# Autodesk Inventor assembly: RobotAsem
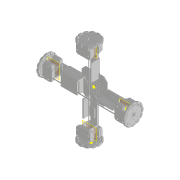
[picture p0: Inventor's stored thumbnail of the model, 180x180]
Saved by Autodesk Inventor 2022 (Build 260153000, 153)
## iProperties
Created: 2022-10-20
Part Number: RobotAsem
Document SubType Name: Assembly
Designer: MVeszpremi
Author: MVeszpremi
## Documents named in this file (8)
- C:\Users\veszp\Dropbox\180DAB CAD\RobotAsem.iam
- C:\Users\veszp\Dropbox\180DAB CAD\RobotBase.ipt
- C:\Users\veszp\Dropbox\180DAB CAD\StepperMotorHolder.ipt
- C:\Users\veszp\Dropbox\180DAB CAD\RobotBaseMotorExt.ipt
- C:\Users\veszp\Dropbox\180DAB CAD\Placeholde_stepperdriverr.ipt
- C:\Users\veszp\Dropbox\180DAB CAD\Wheel.ipt
- C:\Users\veszp\Dropbox\180DAB CAD\BaseStabilizerAttachment.ipt
- C:\Users\veszp\Dropbox\180DAB CAD\Paceholder_shaft.ipt
## Components (20 placed, 7 different names)
1. RobotBase:1 — Mate:1, Mate:2, Mate:3, Mate:4, Mate:5, Mate:6, Mate:7, Mate:8, Mate:9, Mate:10, Mate:11, Mate:12
2. RobotBaseMotorExt:1 — Mate:1, Mate:2, Mate:3, Mate:25, Mate:26, Mate:36, Mate:37, Mate:38
3. RobotBaseMotorExt:2 — Mate:4, Mate:5, Mate:6, Mate:27, Mate:28, Mate:29
4. RobotBaseMotorExt:3 — Mate:7, Mate:8, Mate:9, Mate:33, Mate:34, Mate:35
5. RobotBaseMotorExt:4 — Mate:10, Mate:11, Mate:12, Mate:30, Mate:31, Mate:32
6. Placeholde_stepperdriverr:1 — Mate:25, Mate:26
7. StepperMotorHolder:1 — Mate:27, Mate:28, Mate:29, Mate:43, Mate:44, Mate:45, Mate:46
8. StepperMotorHolder:2 — Mate:30, Mate:31, Mate:32, Mate:41, Mate:47, Mate:48, Mate:49
9. StepperMotorHolder:3 — Mate:33, Mate:34, Mate:35, Mate:42, Mate:50, Mate:51, Mate:52
10. StepperMotorHolder:4 — Mate:36, Mate:37, Mate:38, Mate:39, Mate:40, Mate:53, Mate:54, Mate:55
11. Wheel:1 — Mate:39, Mate:40
12. Wheel:2 — Mate:41
13. Wheel:3 — Mate:42
14. Wheel:4 — Mate:43
15. BaseStabilizerAttachment:1 — Mate:44, Mate:45, Mate:46, Mate:58
16. BaseStabilizerAttachment:2 — Mate:47, Mate:48, Mate:49, Mate:59
17. BaseStabilizerAttachment:3 — Mate:50, Mate:51, Mate:52, Mate:57
18. BaseStabilizerAttachment:4 — Mate:53, Mate:54, Mate:55, Mate:56
19. Paceholder_shaft:1 — Mate:56, Mate:57
20. Paceholder_shaft:2 — Mate:58, Mate:59
## Relationships (47: Mate 47)
- Mate:1: RobotBase:1 ↔ RobotBaseMotorExt:1
- Mate:2: RobotBase:1 ↔ RobotBaseMotorExt:1
- Mate:3: RobotBase:1 ↔ RobotBaseMotorExt:1
- Mate:4: RobotBase:1 ↔ RobotBaseMotorExt:2
- Mate:5: RobotBase:1 ↔ RobotBaseMotorExt:2
- Mate:6: RobotBase:1 ↔ RobotBaseMotorExt:2
- Mate:7: RobotBase:1 ↔ RobotBaseMotorExt:3
- Mate:8: RobotBase:1 ↔ RobotBaseMotorExt:3
- Mate:9: RobotBase:1 ↔ RobotBaseMotorExt:3
- Mate:10: RobotBase:1 ↔ RobotBaseMotorExt:4
- Mate:11: RobotBase:1 ↔ RobotBaseMotorExt:4
- Mate:12: RobotBase:1 ↔ RobotBaseMotorExt:4
- Mate:25: RobotBaseMotorExt:1 ↔ Placeholde_stepperdriverr:1
- Mate:26 (6.5 mm): RobotBaseMotorExt:1 ↔ Placeholde_stepperdriverr:1
- Mate:27: RobotBaseMotorExt:2 ↔ StepperMotorHolder:1
- Mate:28: RobotBaseMotorExt:2 ↔ StepperMotorHolder:1
- Mate:29: RobotBaseMotorExt:2 ↔ StepperMotorHolder:1
- Mate:30: RobotBaseMotorExt:4 ↔ StepperMotorHolder:2
- Mate:31: RobotBaseMotorExt:4 ↔ StepperMotorHolder:2
- Mate:32: RobotBaseMotorExt:4 ↔ StepperMotorHolder:2
- Mate:33: RobotBaseMotorExt:3 ↔ StepperMotorHolder:3
- Mate:34: RobotBaseMotorExt:3 ↔ StepperMotorHolder:3
- Mate:35: RobotBaseMotorExt:3 ↔ StepperMotorHolder:3
- Mate:36: RobotBaseMotorExt:1 ↔ StepperMotorHolder:4
- Mate:37: RobotBaseMotorExt:1 ↔ StepperMotorHolder:4
- Mate:38: RobotBaseMotorExt:1 ↔ StepperMotorHolder:4
- Mate:39: StepperMotorHolder:4 ↔ Wheel:1
- Mate:40 (5.5 mm): StepperMotorHolder:4 ↔ Wheel:1
- Mate:41: StepperMotorHolder:2 ↔ Wheel:2
- Mate:42: StepperMotorHolder:3 ↔ Wheel:3
- Mate:43: StepperMotorHolder:1 ↔ Wheel:4
- Mate:44: StepperMotorHolder:1 ↔ BaseStabilizerAttachment:1
- Mate:45: StepperMotorHolder:1 ↔ BaseStabilizerAttachment:1
- Mate:46: StepperMotorHolder:1 ↔ BaseStabilizerAttachment:1
- Mate:47: StepperMotorHolder:2 ↔ BaseStabilizerAttachment:2
- Mate:48: StepperMotorHolder:2 ↔ BaseStabilizerAttachment:2
- Mate:49: StepperMotorHolder:2 ↔ BaseStabilizerAttachment:2
- Mate:50: StepperMotorHolder:3 ↔ BaseStabilizerAttachment:3
- Mate:51: StepperMotorHolder:3 ↔ BaseStabilizerAttachment:3
- Mate:52: StepperMotorHolder:3 ↔ BaseStabilizerAttachment:3
- Mate:53: StepperMotorHolder:4 ↔ BaseStabilizerAttachment:4
- Mate:54: StepperMotorHolder:4 ↔ BaseStabilizerAttachment:4
- Mate:55: StepperMotorHolder:4 ↔ BaseStabilizerAttachment:4
- Mate:56: BaseStabilizerAttachment:4 ↔ Paceholder_shaft:1
- Mate:57: BaseStabilizerAttachment:3 ↔ Paceholder_shaft:1
- Mate:58: BaseStabilizerAttachment:1 ↔ Paceholder_shaft:2
- Mate:59: BaseStabilizerAttachment:2 ↔ Paceholder_shaft:2
